# Autodesk Inventor assembly: Caja motriz 2b_CasaCentral
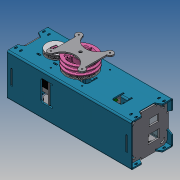
[picture p0: Inventor's stored thumbnail of the model, 180x180]
Saved by Autodesk Inventor 2017 (Build 210142000, 142)
## iProperties
Part Number: Caja motriz 2b_CasaCentral
Material: Genérico
Document SubType Name: Assembly
Designer: leo
Author: FABLAB
## Documents named in this file (7)
- C:\Users\Leo\Documents\GitHub\actor-re-actor\models\inventor-caja\Caja motriz 2b_CasaCentral.iam
- C:\Users\Leo\Documents\GitHub\actor-re-actor\models\inventor-caja\ensamble caja motriz\Design Accelerator\Conexión por perno1.iam
- C:\Users\Leo\Documents\GitHub\actor-re-actor\models\inventor-caja\ensamble caja motriz\Design Accelerator\Conexión por perno2.iam
- C:\Users\Leo\Documents\GitHub\actor-re-actor\models\inventor-caja\Piezas\componentes.iam
- C:\Users\Leo\Documents\GitHub\actor-re-actor\models\inventor-caja\Case\Case-D.iam
- C:\Users\Leo\Documents\GitHub\actor-re-actor\models\inventor-caja\partes transmision\conjunto polea plato-carrete.iam
- C:\Users\Leo\Documents\GitHub\actor-re-actor\models\inventor-caja\partes transmision\Potencia2.iam
## Components (6 placed, 5 different names)
1. Case-D:1 [sub-assembly] — Coincidencia:1, Coincidencia:4, Coincidencia:9, Nivelación:12, Coincidencia:11, Coincidencia:12, Coincidencia:13, Nivelación:13
2. Potencia2:1 [sub-assembly] — Coincidencia:1, Coincidencia:2, Coincidencia:3, Coincidencia:10
3. conjunto polea plato-carrete:1 [sub-assembly] — Coincidencia:4, Coincidencia:5, Coincidencia:6
4. Conexión por perno:1 [sub-assembly] — Coincidencia:12, Coincidencia:13
5. Conexión por perno:2 [sub-assembly] — Coincidencia:9, Coincidencia:10
6. componentes:1 [sub-assembly] — Nivelación:12, Coincidencia:11, Nivelación:13
## Relationships (13: Mate 11, Flush 2)
- Coincidencia:1 [Mate]: Case-D:1 ↔ Potencia2:1
- Coincidencia:2 [Mate]: Potencia2:1
- Coincidencia:3 [Mate]: Potencia2:1
- Coincidencia:4 [Mate] (5 mm): Case-D:1 ↔ conjunto polea plato-carrete:1
- Coincidencia:5 [Mate]: conjunto polea plato-carrete:1
- Coincidencia:6 [Mate] (72 mm): conjunto polea plato-carrete:1
- Coincidencia:9 [Mate]: Case-D:1 ↔ Conexión por perno:2
- Coincidencia:10 [Mate]: Potencia2:1 ↔ Conexión por perno:2
- Nivelación:12 [Flush]: Case-D:1 ↔ componentes:1
- Coincidencia:11 [Mate]: Case-D:1 ↔ componentes:1
- Coincidencia:12 [Mate]: Case-D:1 ↔ Conexión por perno:1
- Coincidencia:13 [Mate]: Case-D:1 ↔ Conexión por perno:1
- Nivelación:13 [Flush]: Case-D:1 ↔ componentes:1
